# Autodesk Inventor assembly: BulletHolderAssembly
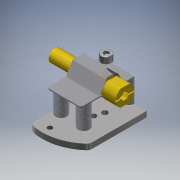
[picture p0: Inventor's stored thumbnail of the model, 180x180]
Saved by Autodesk Inventor 2019 (Build 230136000, 136)
## iProperties
Created: 2018-08-03
Part Number: BulletHolderAssembly
Document SubType Name: Assembly
Designer: Sergey
Author: Sergey
## Documents named in this file (7)
- C:\Users\user\Documents\Inventor@SVN\Moore Scienta DA30 system\e-beam-heater-Moore\BulletHolderAssembly.iam
- C:\Users\user\Documents\Inventor@SVN\Moore Scienta DA30 system\e-beam-heater-Moore\ANSI B18.3 - 6-40 UNF - 0.25(31).ipt
- C:\Users\user\Documents\Inventor@SVN\Moore Scienta DA30 system\e-beam-heater-Moore\Bullet_v5_SiliconeSample_Assembly.iam
- C:\Users\user\Documents\Inventor@SVN\Moore Scienta DA30 system\e-beam-heater-Moore\Bullet_Holder_SheetMetal_v6.ipt
- C:\Users\user\Documents\Inventor@SVN\Moore Scienta DA30 system\e-beam-heater-Moore\BulletHolderSpring_v1.ipt
- C:\Users\user\Documents\Inventor@SVN\Moore Scienta DA30 system\e-beam-heater-Moore\Shield_3_Ground_v4.ipt
- C:\Users\user\Documents\Inventor@SVN\Moore Scienta DA30 system\e-beam-heater-Moore\Standoff.ipt
## Components (11 placed, 6 different names)
1. Shield_3_Ground_v4:1 — Flush:1, Flush:2, Flush:3, Mate:1, Mate:2, Mate:3, Mate:4, Mate:5, Mate:6, Mate:7, Mate:8, Mate:11, Mate:12, Mate:14, Flush:4
2. Hexagon Socket Head Cap Screw - Inch 6-40 UNF - 0.25:1 — Mate:1, Mate:4, Mate:10
3. Hexagon Socket Head Cap Screw - Inch 6-40 UNF - 0.25:2 — Mate:2, Mate:3, Mate:9
4. Bullet_v5_SiliconeSample_Assembly:1 [sub-assembly] — Mate:19, Mate:20
5. Standoff:9 — Mate:6, Mate:10
6. Standoff:10 — Mate:5, Mate:9, Mate:13, Mate:18
7. Standoff:11 — Mate:7, Mate:11
8. Standoff:12 — Mate:8, Mate:12
9. Bullet_Holder_SheetMetal_v6:1 — Mate:13, Mate:14, Flush:4, Mate:19, Mate:20, Mate:21
10. BulletHolderSpring_v1:1 — Mate:21, Mate:22
11. Hexagon Socket Head Cap Screw - Inch 6-40 UNF - 0.25:3 — Mate:18, Mate:22
## Relationships (23: Mate 19, Flush 4)
- Flush:1: Shield_3_Ground_v4:1
- Flush:2: Shield_3_Ground_v4:1
- Flush:3: Shield_3_Ground_v4:1
- Mate:1: Shield_3_Ground_v4:1 ↔ Hexagon Socket Head Cap Screw - Inch 6-40 UNF - 0.25:1
- Mate:2: Shield_3_Ground_v4:1 ↔ Hexagon Socket Head Cap Screw - Inch 6-40 UNF - 0.25:2
- Mate:3: Shield_3_Ground_v4:1 ↔ Hexagon Socket Head Cap Screw - Inch 6-40 UNF - 0.25:2
- Mate:4: Shield_3_Ground_v4:1 ↔ Hexagon Socket Head Cap Screw - Inch 6-40 UNF - 0.25:1
- Mate:5: Shield_3_Ground_v4:1 ↔ Standoff:10
- Mate:6: Shield_3_Ground_v4:1 ↔ Standoff:9
- Mate:7: Shield_3_Ground_v4:1 ↔ Standoff:11
- Mate:8: Shield_3_Ground_v4:1 ↔ Standoff:12
- Mate:9: Hexagon Socket Head Cap Screw - Inch 6-40 UNF - 0.25:2 ↔ Standoff:10
- Mate:10: Hexagon Socket Head Cap Screw - Inch 6-40 UNF - 0.25:1 ↔ Standoff:9
- Mate:11: Shield_3_Ground_v4:1 ↔ Standoff:11
- Mate:12: Shield_3_Ground_v4:1 ↔ Standoff:12
- Mate:13: Standoff:10 ↔ Bullet_Holder_SheetMetal_v6:1
- Mate:14: Shield_3_Ground_v4:1 ↔ Bullet_Holder_SheetMetal_v6:1
- Flush:4 (0.635 mm): Shield_3_Ground_v4:1 ↔ Bullet_Holder_SheetMetal_v6:1
- Mate:18: Standoff:10 ↔ Hexagon Socket Head Cap Screw - Inch 6-40 UNF - 0.25:3
- Mate:19: Bullet_v5_SiliconeSample_Assembly:1 ↔ Bullet_Holder_SheetMetal_v6:1
- Mate:20: Bullet_v5_SiliconeSample_Assembly:1 ↔ Bullet_Holder_SheetMetal_v6:1
- Mate:21: Bullet_Holder_SheetMetal_v6:1 ↔ BulletHolderSpring_v1:1
- Mate:22: BulletHolderSpring_v1:1 ↔ Hexagon Socket Head Cap Screw - Inch 6-40 UNF - 0.25:3
